# Autodesk Inventor assembly: assembly
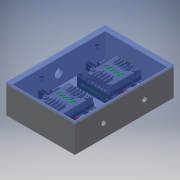
[picture p0: Inventor's stored thumbnail of the model, 180x180]
Saved by Autodesk Inventor 2017 SP1 (Build 210196100, 196)
## iProperties
Created: 2016-12-24
Part Number: assembly
Document SubType Name: Assembly
Designer: wsh32
Author: wsh32
## Documents named in this file (4)
- C:\Users\wsh32\Documents\Inventor\ControlBox\assembly.iam
- C:\Users\wsh32\Documents\Inventor\ControlBox\bottom.ipt
- C:\Users\wsh32\Documents\Inventor\ControlBox\top.ipt
- C:\Users\wsh32\Documents\Inventor\ControlBox\talon.ipt
## Components (4 placed, 3 different names)
1. bottom:1 — Mate:1, Mate:2, Mate:5, Mate:6, Mate:7, Flush:1, Mate:8, Mate:9, Flush:2
2. top:1 — Mate:7, Flush:1, Flush:2
3. talon:1 — Mate:1, Mate:8, Mate:9
4. talon:2 — Mate:2, Mate:5, Mate:6
## Relationships (9: Mate 7, Flush 2)
- Mate:1: bottom:1 ↔ talon:1
- Mate:2: bottom:1 ↔ talon:2
- Mate:5: bottom:1 ↔ talon:2
- Mate:6: bottom:1 ↔ talon:2
- Mate:7: bottom:1 ↔ top:1
- Flush:1: bottom:1 ↔ top:1
- Mate:8: bottom:1 ↔ talon:1
- Mate:9: bottom:1 ↔ talon:1
- Flush:2: bottom:1 ↔ top:1
